# Autodesk Inventor assembly: CE-5.2.3
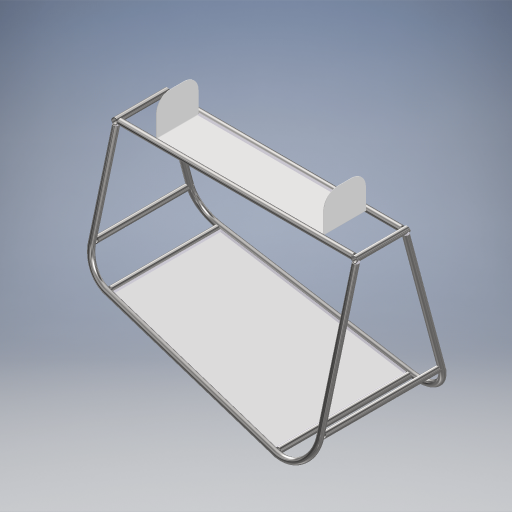
[picture p0: Inventor's stored thumbnail of the model, 512x512]
Saved by Autodesk Inventor 2024 (Build 280153000, 153)
## iProperties
_SolveAssemblyDoc: Frame Generator Solve Assembly
_Version: 25.0.0
Created: 2024-02-15
Part Number: CE-5.2.3
Document SubType Name: Weldment
Designer: Alex
Weld Material: Welded Aluminum-6061
Author: Alex
## Documents named in this file (5)
- C:\Shared\alex-bartella-schoolwork\4z03\Week 5\CE-5.2.3.iam
- C:\Shared\alex-bartella-schoolwork\4z03\Week 5\CE-5.2.3-01-WF.ipt
- C:\Shared\alex-bartella-schoolwork\4z03\Week 5\CE-5.2.3\Frame\CE-5.2.3-01.iam
- C:\Shared\alex-bartella-schoolwork\4z03\Week 5\CE-5.2.3\Frame\CE-5.2.3-02.ipt
- C:\Shared\alex-bartella-schoolwork\4z03\Week 5\CE-5.2.3\Frame\CE-5.2.3-03.ipt
## Components (4 placed, 4 different names)
1. CE-5.2.3-01-WF:1 — Flush:2, Flush:3
2. CE-5.2.3-01:1 [sub-assembly]
3. CE-5.2.3-02:1 — Flush:2
4. CE-5.2.3-03:1 — Flush:3
## Relationships (2: Flush 2)
- Flush:2: CE-5.2.3-01-WF:1 ↔ CE-5.2.3-02:1
- Flush:3: CE-5.2.3-01-WF:1 ↔ CE-5.2.3-03:1
